# Autodesk Inventor assembly: DriveTrainMotor+Mount
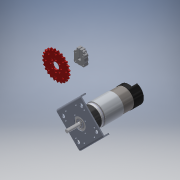
[picture p0: Inventor's stored thumbnail of the model, 180x180]
Saved by Autodesk Inventor 2018 (Build 220112000, 112)
## iProperties
Created: 2017-11-14
Part Number: DriveTrainMotor+Mount
Document SubType Name: Assembly
Designer: ball
Author: ball
## Documents named in this file (5)
- C:\FTC\2017Robot\DriveTrainMotor+Mount.iam
- C:\FTC\Andymark\am-3461a+NeveRest+Orbital+3.7+REV2.ipt
- C:\FTC\Andymark\am-3474 actobotics hole pattern.ipt
- C:\FTC\Actobotics\615 parts\615106.ipt
- C:\FTC\Actobotics\545 parts\545618 assembly.ipt
## Components (4 placed, 4 different names)
1. am-3461a+NeveRest+Orbital+3.7+REV2:1 — Mate:1, Mate:2, Mate:3, Mate:4
2. am-3474 actobotics hole pattern:2 — Mate:1, Mate:2, Mate:3, Mate:4
3. 615106:1
4. 545618 assembly:1
## Relationships (4: Mate 4)
- Mate:1: am-3461a+NeveRest+Orbital+3.7+REV2:1 ↔ am-3474 actobotics hole pattern:2
- Mate:2: am-3461a+NeveRest+Orbital+3.7+REV2:1 ↔ am-3474 actobotics hole pattern:2
- Mate:3: am-3461a+NeveRest+Orbital+3.7+REV2:1 ↔ am-3474 actobotics hole pattern:2
- Mate:4: am-3461a+NeveRest+Orbital+3.7+REV2:1 ↔ am-3474 actobotics hole pattern:2
